# Autodesk Inventor assembly: Assembly_Cube_Z-Focus_Linearbearing_mechanical_1x1_v3
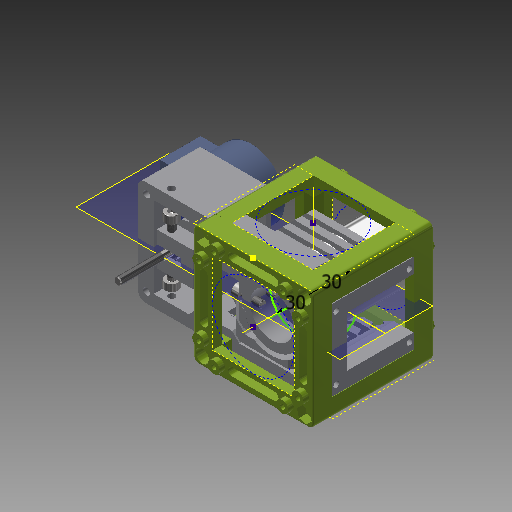
[picture p0: Inventor's stored thumbnail of the model, 512x512]
Saved by Autodesk Inventor 2019 (Build 230136000, 136)
## iProperties
Created: 2020-07-30
Part Number: Assembly_Cube_Z-Focus_Linearbearing_mechanical_1x1_v3
Document SubType Name: Assembly
Designer: marsikovabarbora
Author: marsikovabarbora
## Documents named in this file (10)
- C:\Users\marsikovabarbora\Dropbox\UC2\02_CAD\INVENTOR\uc2_v3\Assembly_Cube_Z-Focus_Linearbearing_motorized_small_1x1_v3.iam
- C:\Users\marsikovabarbora\Dropbox\UC2\02_CAD\INVENTOR\uc2_v3\Assembly_Cube_empty_IM_v3.iam
- C:\Users\marsikovabarbora\Documents\Inventor\Content Center Files\R2019\en-US\DIN 912\DIN 912 - M3 x 0,5 x 30 x 18.ipt
- C:\Users\marsikovabarbora\Documents\Inventor\Content Center Files\R2019\en-US\DIN 912\DIN 912 - M3 x 0,5 x 8 x 6,75.ipt
- C:\Users\marsikovabarbora\Dropbox\UC2\02_CAD\INVENTOR\uc2_v3\20_focus_inlet_objective_mount_v8.ipt
- C:\Users\marsikovabarbora\Dropbox\UC2\02_CAD\INVENTOR\uc2_v3\00_Microscope_Objective_Lens10x.ipt
- C:\Users\marsikovabarbora\Documents\Inventor\Content Center Files\R2019\en-US\DIN 934\DIN 934 - M3 x 0,5.ipt
- C:\Users\marsikovabarbora\Dropbox\UC2\02_CAD\INVENTOR\uc2_v3\20_focus_inlet_linearflexure_motorized_small_v3.ipt
- C:\Users\marsikovabarbora\Dropbox\UC2\02_CAD\INVENTOR\uc2_v3\00_Stepper_Motor_28BYJ-48.ipt
- C:\Users\marsikovabarbora\Dropbox\UC2\02_CAD\INVENTOR\uc2_v3\30_Coupling_Screw_28BYJ_M3.ipt
## Components (12 placed, 9 different names)
1. Assembly_Cube_empty_IM_v3:1 [sub-assembly] — Mate:1, Mate:2, Flush:1, Mate:27, Flush:5, Flush:6, Angle:1
2. 20_focus_inlet_linearflexure_motorized_small_v3:1 — Mate:8, Mate:15, Mate:16, Passend:21, Passend:23, Fluchtend:3, Mate:27, Flush:5, Flush:6, Flush:9, Flush:10, Mate:30
3. DIN 912 - replaced by DIN EN ISO 4762 M3 x 30:1 — Passend:25, Mate:29, Flush:8, Mate:30
4. DIN 912 - replaced by DIN EN ISO 4762 M3 x 8:1 — Mate:15, Mate:32
5. DIN 912 - replaced by DIN EN ISO 4762 M3 x 8:2 — Mate:16, Mate:31
6. DIN 912 - replaced by DIN EN ISO 4762 M3 x 8:3 — Mate:8, Passend:19, Fluchtend:2
7. 20_focus_inlet_objective_mount_v8:1 — Mate:18, Passend:19, Passend:20, Passend:21, Passend:22, Fluchtend:3
8. 00_Microscope_Objective_Lens10x:1 — Mate:18, Passend:22
9. DIN 912 - replaced by DIN EN ISO 4762 M3 x 8:5 — Passend:20, Fluchtend:2, Passend:23
10. DIN 934 - replaced by DIN EN 24032/28673/28674 M3:1 — Passend:25, Mate:31, Mate:32
11. 00_Stepper_Motor_28BYJ-48:1 — Mate:28, Flush:7, Flush:9, Angle:1, Flush:10
12. 30_Coupling_Screw_28BYJ_M3:1 — Mate:28, Flush:7, Mate:29, Flush:8
## Relationships (28: Mate 18, Flush 9, Angle 1)
- Mate:1: Assembly_Cube_empty_IM_v3:1
- Mate:2: Assembly_Cube_empty_IM_v3:1
- Flush:1: Assembly_Cube_empty_IM_v3:1
- Mate:8: 20_focus_inlet_linearflexure_motorized_small_v3:1 ↔ DIN 912 - replaced by DIN EN ISO 4762 M3 x 8:3
- Mate:15: 20_focus_inlet_linearflexure_motorized_small_v3:1 ↔ DIN 912 - replaced by DIN EN ISO 4762 M3 x 8:1
- Mate:16: 20_focus_inlet_linearflexure_motorized_small_v3:1 ↔ DIN 912 - replaced by DIN EN ISO 4762 M3 x 8:2
- Mate:18: 20_focus_inlet_objective_mount_v8:1 ↔ 00_Microscope_Objective_Lens10x:1
- Passend:19 [Mate]: DIN 912 - replaced by DIN EN ISO 4762 M3 x 8:3 ↔ 20_focus_inlet_objective_mount_v8:1
- Passend:20 [Mate]: 20_focus_inlet_objective_mount_v8:1 ↔ DIN 912 - replaced by DIN EN ISO 4762 M3 x 8:5
- Fluchtend:2 [Flush]: DIN 912 - replaced by DIN EN ISO 4762 M3 x 8:3 ↔ DIN 912 - replaced by DIN EN ISO 4762 M3 x 8:5
- Passend:21 [Mate]: 20_focus_inlet_linearflexure_motorized_small_v3:1 ↔ 20_focus_inlet_objective_mount_v8:1
- Passend:22 [Mate]: 20_focus_inlet_objective_mount_v8:1 ↔ 00_Microscope_Objective_Lens10x:1
- Passend:23 [Mate]: 20_focus_inlet_linearflexure_motorized_small_v3:1 ↔ DIN 912 - replaced by DIN EN ISO 4762 M3 x 8:5
- Fluchtend:3 [Flush]: 20_focus_inlet_linearflexure_motorized_small_v3:1 ↔ 20_focus_inlet_objective_mount_v8:1
- Passend:25 [Mate]: DIN 912 - replaced by DIN EN ISO 4762 M3 x 30:1 ↔ DIN 934 - replaced by DIN EN 24032/28673/28674 M3:1
- Mate:27: Assembly_Cube_empty_IM_v3:1 ↔ 20_focus_inlet_linearflexure_motorized_small_v3:1
- Flush:5: Assembly_Cube_empty_IM_v3:1 ↔ 20_focus_inlet_linearflexure_motorized_small_v3:1
- Flush:6: Assembly_Cube_empty_IM_v3:1 ↔ 20_focus_inlet_linearflexure_motorized_small_v3:1
- Mate:28: 00_Stepper_Motor_28BYJ-48:1 ↔ 30_Coupling_Screw_28BYJ_M3:1
- Flush:7: 00_Stepper_Motor_28BYJ-48:1 ↔ 30_Coupling_Screw_28BYJ_M3:1
- Mate:29: DIN 912 - replaced by DIN EN ISO 4762 M3 x 30:1 ↔ 30_Coupling_Screw_28BYJ_M3:1
- Flush:8: DIN 912 - replaced by DIN EN ISO 4762 M3 x 30:1 ↔ 30_Coupling_Screw_28BYJ_M3:1
- Flush:9: 20_focus_inlet_linearflexure_motorized_small_v3:1 ↔ 00_Stepper_Motor_28BYJ-48:1
- Angle:1 (180 deg): Assembly_Cube_empty_IM_v3:1 ↔ 00_Stepper_Motor_28BYJ-48:1
- Flush:10: 20_focus_inlet_linearflexure_motorized_small_v3:1 ↔ 00_Stepper_Motor_28BYJ-48:1
- Mate:30: 20_focus_inlet_linearflexure_motorized_small_v3:1 ↔ DIN 912 - replaced by DIN EN ISO 4762 M3 x 30:1
- Mate:31: DIN 912 - replaced by DIN EN ISO 4762 M3 x 8:2 ↔ DIN 934 - replaced by DIN EN 24032/28673/28674 M3:1
- Mate:32: DIN 912 - replaced by DIN EN ISO 4762 M3 x 8:1 ↔ DIN 934 - replaced by DIN EN 24032/28673/28674 M3:1
